# Autodesk Inventor assembly: LampeSolaire2
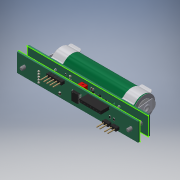
[picture p0: Inventor's stored thumbnail of the model, 180x180]
Saved by Autodesk Inventor 2019 (Build 230136000, 136)
## iProperties
Created: 2020-09-14
Part Number: LampeSolaire2
Document SubType Name: Assembly
Designer: nicolas
Author: nicolas
## Documents named in this file (4)
- C:\Workspace\3D\Autodesk\Projects\LampeSolaire2\LampeSolaire2.iam
- C:\Workspace\3D\Cad\ChargerModule.ipt
- C:\Workspace\3D\Cad\LampeSolaire2.ipt
- C:\Workspace\3D\Autodesk\Parts\Screws\92949A329_18-8 SS BUTTON HEAD HEX DRIVE SCREW.ipt
## Components (4 placed, 3 different names)
1. ChargerModule:1 — Flush:1, Flush:2, Mate:1, Cylindrical:1, Cylindrical:2, Mate:2, Mate:3
2. LampeSolaire2:1 — Flush:1, Flush:2, Mate:1
3. 92949A329_18-8 SS BUTTON HEAD HEX DRIVE SCREW:1 — Cylindrical:1, Mate:3
4. 92949A329_18-8 SS BUTTON HEAD HEX DRIVE SCREW:2 — Cylindrical:2, Mate:2
## Relationships (7: Mate 3, Flush 2, CylindricalJoint 2)
- Flush:1: ChargerModule:1 ↔ LampeSolaire2:1
- Flush:2: ChargerModule:1 ↔ LampeSolaire2:1
- Mate:1: ChargerModule:1 ↔ LampeSolaire2:1
- Cylindrical:1: ChargerModule:1 ↔ 92949A329_18-8 SS BUTTON HEAD HEX DRIVE SCREW:1
- Cylindrical:2: ChargerModule:1 ↔ 92949A329_18-8 SS BUTTON HEAD HEX DRIVE SCREW:2
- Mate:2: ChargerModule:1 ↔ 92949A329_18-8 SS BUTTON HEAD HEX DRIVE SCREW:2
- Mate:3: ChargerModule:1 ↔ 92949A329_18-8 SS BUTTON HEAD HEX DRIVE SCREW:1
